# Autodesk Inventor assembly: MotorsAndBase
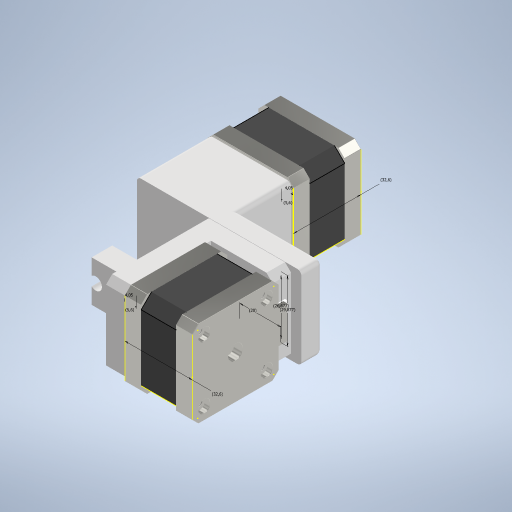
[picture p0: Inventor's stored thumbnail of the model, 512x512]
Saved by Autodesk Inventor 2024 (Build 280153000, 153)
## iProperties
Created: 2025-05-07
Part Number: MotorsAndBase
Document SubType Name: Assembly
Designer: Bjarni Heselmans
Author: Bjarni Heselmans
## Documents named in this file (5)
- C:\Users\Bjarni Heselmans\Desktop\Cursussen\2024-2025\Project Engeneering\2EAI-POE-SpotNShot\docs\3D-Files\MotorsAndBase.iam
- C:\Users\Bjarni Heselmans\Desktop\Cursussen\2024-2025\Project Engeneering\2EAI-POE-SpotNShot\docs\3D-Files\afterdesign.ipt
- C:\Users\Bjarni Heselmans\Desktop\Cursussen\2024-2025\Project Engeneering\2EAI-POE-SpotNShot\docs\3D-Files\NEMA_17.ipt
- C:\Users\Bjarni Heselmans\Desktop\Cursussen\2024-2025\Project Engeneering\2EAI-POE-SpotNShot\docs\3D-Files\MotorMount.ipt
- C:\Users\Bjarni Heselmans\Desktop\Cursussen\2024-2025\Project Engeneering\2EAI-POE-SpotNShot\docs\3D-Files\LazerMount.ipt
## Components (5 placed, 4 different names)
1. afterdesign:1 — Mate:3, Mate:4, Mate:5, Mate:6, Mate:7
2. NEMA_17:2 — Mate:3, Mate:4
3. MotorMount:1 — Mate:5, Mate:6, Mate:7, Mate:8, Mate:9
4. NEMA_17:3 — Mate:8, Mate:9, Mate:10, Mate:11
5. LazerMount:1 — Mate:10, Mate:11
## Relationships (9: Mate 9)
- Mate:3: afterdesign:1 ↔ NEMA_17:2
- Mate:4: afterdesign:1 ↔ NEMA_17:2
- Mate:5: afterdesign:1 ↔ MotorMount:1
- Mate:6: afterdesign:1 ↔ MotorMount:1
- Mate:7: afterdesign:1 ↔ MotorMount:1
- Mate:8: MotorMount:1 ↔ NEMA_17:3
- Mate:9: MotorMount:1 ↔ NEMA_17:3
- Mate:10: NEMA_17:3 ↔ LazerMount:1
- Mate:11: NEMA_17:3 ↔ LazerMount:1
